# Autodesk Inventor assembly: Worm shaft tilting head - gripper
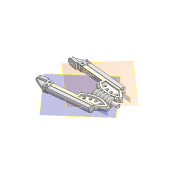
[picture p0: Inventor's stored thumbnail of the model, 180x180]
Saved by Autodesk Inventor 2020.3 (Build 243373010, 373A)
## iProperties
Created: 2021-05-15
Part Number: Worm shaft tilting head - gripper
Document SubType Name: Assembly
Designer: marti
Author: marti
## Documents named in this file (5)
- C:\Users\marti\Documents\Inventor\RobotManipulateArm\17.4.2021 - Complete new IDEA\Worm shaft tilting head - gripper.iam
- C:\Users\marti\Documents\Inventor\RobotManipulateArm\17.4.2021 - Complete new IDEA\Worm shaft tilting head - gripper\Design Accelerator\Worm Gears1.iam
- C:\Users\marti\Documents\Inventor\RobotManipulateArm\17.4.2021 - Complete new IDEA\Holder of gripper.ipt
- C:\Users\marti\Documents\Inventor\RobotManipulateArm\17.4.2021 - Complete new IDEA\Second part of arm of gripper.ipt
- C:\Users\marti\Documents\Inventor\RobotManipulateArm\17.4.2021 - Complete new IDEA\Worm shaft tilting head - gripper\Design Accelerator\Worm Gears1_MIR.iam
## Components (6 placed, 4 different names)
1. Worm Gears:1 [sub-assembly] — Mate:1, Mate:2, Angle:1, Angle:2, Angle:4
2. Holder of gripper:1 — Mate:1, Mate:2, Mate:3, Mate:4, Angle:2
3. Second part of arm of gripper:1 — Mate:3, Mate:4, Angle:4
4. Worm Gears1_MIR:1 [sub-assembly] — Mate:5, Mate:6, Angle:3
5. Holder of gripper:2 — Mate:5, Mate:6, Mate:7, Mate:8, Angle:1
6. Second part of arm of gripper:2 — Mate:7, Mate:8, Angle:3
## Relationships (12: Mate 8, Angle 4)
- Mate:1: Worm Gears:1 ↔ Holder of gripper:1
- Mate:2: Worm Gears:1 ↔ Holder of gripper:1
- Mate:3: Holder of gripper:1 ↔ Second part of arm of gripper:1
- Mate:4: Holder of gripper:1 ↔ Second part of arm of gripper:1
- Mate:5: Worm Gears1_MIR:1 ↔ Holder of gripper:2
- Mate:6: Worm Gears1_MIR:1 ↔ Holder of gripper:2
- Mate:7: Holder of gripper:2 ↔ Second part of arm of gripper:2
- Mate:8: Holder of gripper:2 ↔ Second part of arm of gripper:2
- Angle:1 (-10 deg): Worm Gears:1 ↔ Holder of gripper:2
- Angle:2 (170 deg): Worm Gears:1 ↔ Holder of gripper:1
- Angle:3 (180 deg): Worm Gears1_MIR:1 ↔ Second part of arm of gripper:2
- Angle:4 (180 deg): Worm Gears:1 ↔ Second part of arm of gripper:1
